# Autodesk Inventor assembly: Ensamblaje2
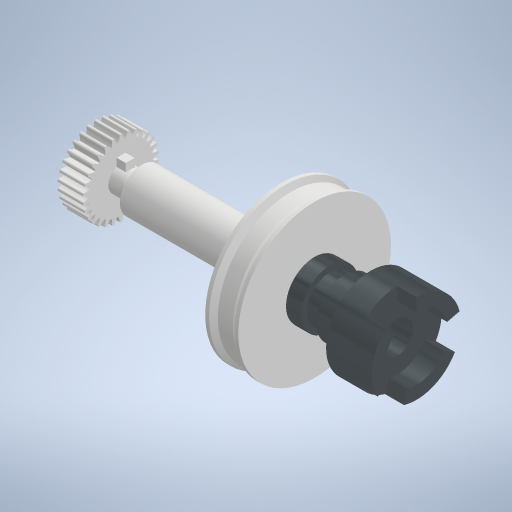
[picture p0: Inventor's stored thumbnail of the model, 512x512]
Saved by Autodesk Inventor 2024.2 (Build 282272000, 272)
## iProperties
Created: 2024-03-20
Part Number: Ensamblaje2
Document SubType Name: Assembly
Designer: Usuario
Author: Usuario
## Documents named in this file (6)
- C:\Users\Usuario\Documents\Vanessa\Ensamblaje2.iam
- C:\Users\Usuario\Downloads\POLEA (1).ipt
- C:\Users\Usuario\Downloads\EJE_CUÑEROS (1).ipt
- C:\Users\Usuario\Downloads\ENGRANE (1).ipt
- C:\Users\Usuario\Downloads\CUÑA (1).ipt
- C:\Users\Usuario\Downloads\tarea 3 dinamica.ipt
## Components (6 placed, 5 different names)
1. POLEA (1):1 — Cilíndrica:1, Nivelación:1
2. EJE_CUÑEROS (1):1 — Cilíndrica:1, Nivelación:1, De rotación:1, Nivelación:2, Rígido:1, Rígido:2, Rígido:3
3. ENGRANE (1):1 — De rotación:1, Nivelación:2
4. CUÑA (1):1 — Rígido:1
5. CUÑA (1):2 — Rígido:2
6. tarea 3 dinamica:1 — Rígido:3
## Relationships (7: WeldJoint 3, Flush 2, CylindricalJoint 1, RevoluteJoint 1)
- Cilíndrica:1 [CylindricalJoint]: POLEA (1):1 ↔ EJE_CUÑEROS (1):1
- Nivelación:1 [Flush]: POLEA (1):1 ↔ EJE_CUÑEROS (1):1
- De rotación:1 [RevoluteJoint]: EJE_CUÑEROS (1):1 ↔ ENGRANE (1):1
- Nivelación:2 [Flush]: EJE_CUÑEROS (1):1 ↔ ENGRANE (1):1
- Rígido:1 [WeldJoint]: EJE_CUÑEROS (1):1 ↔ CUÑA (1):1
- Rígido:2 [WeldJoint]: EJE_CUÑEROS (1):1 ↔ CUÑA (1):2
- Rígido:3 [WeldJoint]: EJE_CUÑEROS (1):1 ↔ tarea 3 dinamica:1
